# Autodesk Inventor assembly: Drivetrain 2025-2026
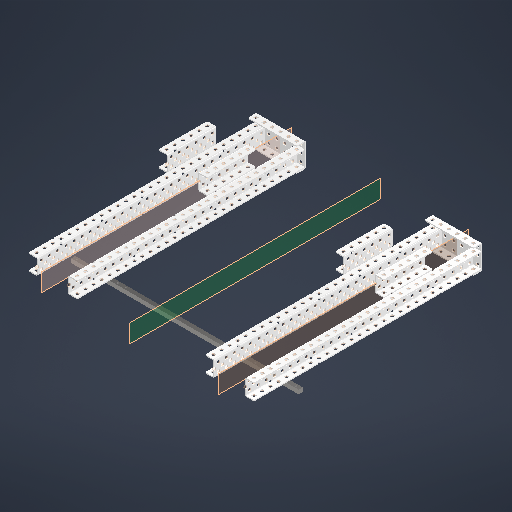
[picture p0: Inventor's stored thumbnail of the model, 512x512]
Saved by Autodesk Inventor 2026.2 (Build 302298000, 298)
## iProperties
Created: 2025-11-06
Part Number: Drivetrain 2025-2026
Document SubType Name: Assembly
Designer: thero
Author: thero
## Documents named in this file (12)
- C:\GitHub Repos\VEX-PushBack_2025-26\Push Back CAD\Drivetrain 2025-2026.iam
- C:\Users\thero\OneDrive\Desktop\VEX-CAD-Inventor-main\Structure\C Channel\Aluminum 1x2x1\Alu C 1x2x1x28.ipt
- C:\Users\thero\OneDrive\Desktop\VEX-CAD-Inventor-main\Structure\C Channel\Aluminum 1x2x1\Alu C 1x2x1x28_MIR.ipt
- C:\Users\thero\OneDrive\Desktop\VEX-CAD-Inventor-main\Structure\C Channel\Aluminum 1x3x1\Alu C 1x3x1x6.ipt
- C:\Users\thero\OneDrive\Desktop\VEX-CAD-Inventor-main\Structure\C Channel\Aluminum 1x2x1\Alu C 1x2x1x6.ipt
- C:\Users\thero\OneDrive\Desktop\VEX-CAD-Inventor-main\Structure\C Channel\Aluminum 1x2x1\Alu C 1x2x1x6_MIR.ipt
- C:\Users\thero\OneDrive\Desktop\VEX-CAD-Inventor-main\Structure\C Channel\Aluminum 1x2x1\Alu C 1x2x1x28_MIR1.ipt
- C:\Users\thero\OneDrive\Desktop\VEX-CAD-Inventor-main\Structure\C Channel\Aluminum 1x2x1\Alu C 1x2x1x28_MIR_MIR.ipt
- C:\Users\thero\OneDrive\Desktop\VEX-CAD-Inventor-main\Structure\C Channel\Aluminum 1x3x1\Alu C 1x3x1x6_MIR.ipt
- C:\Users\thero\OneDrive\Desktop\VEX-CAD-Inventor-main\Structure\C Channel\Aluminum 1x2x1\Alu C 1x2x1x6_MIR1.ipt
- C:\Users\thero\OneDrive\Desktop\VEX-CAD-Inventor-main\Structure\C Channel\Aluminum 1x2x1\Alu C 1x2x1x6_MIR_MIR.ipt
- C:\GitHub Repos\VEX-PushBack_2025-26\Push Back CAD\Chassis Cross Brace.ipt
## Components (11 placed, 11 different names)
1. Alu C 1x2x1x28:1 — Flush:1, Insert:1, Insert:3, Insert:4, Flush:2
2. Alu C 1x2x1x28_MIR:1 — Mate:1, Insert:2, Insert:9
3. Alu C 1x3x1x6:1 — Insert:1, Insert:2
4. Alu C 1x2x1x6:1 — Insert:3, Insert:4
5. Alu C 1x2x1x6_MIR:1
6. Alu C 1x2x1x28_MIR1:1 — Flush:3, Insert:6, Insert:7, Insert:8, Mate:3
7. Alu C 1x2x1x28_MIR_MIR:1 — Mate:2, Insert:5
8. Alu C 1x3x1x6_MIR:1 — Insert:5, Insert:6
9. Alu C 1x2x1x6_MIR1:1 — Insert:7, Insert:8
10. Alu C 1x2x1x6_MIR_MIR:1
11. Chassis Cross Brace:1 — Insert:9
## Relationships (15: Insert 9, Flush 3, Mate 3)
- Flush:1 (-38.1 mm): Alu C 1x2x1x28:1
- Mate:1 (-38.1 mm): Alu C 1x2x1x28_MIR:1
- Insert:1: Alu C 1x2x1x28:1 ↔ Alu C 1x3x1x6:1
- Insert:2: Alu C 1x2x1x28_MIR:1 ↔ Alu C 1x3x1x6:1
- Insert:3 (12.7 mm): Alu C 1x2x1x28:1 ↔ Alu C 1x2x1x6:1
- Insert:4 (12.7 mm): Alu C 1x2x1x28:1 ↔ Alu C 1x2x1x6:1
- Flush:2 (-114.3 mm): Alu C 1x2x1x28:1
- Flush:3 (-38.1 mm): Alu C 1x2x1x28_MIR1:1
- Mate:2 (-38.1 mm): Alu C 1x2x1x28_MIR_MIR:1
- Insert:5: Alu C 1x2x1x28_MIR_MIR:1 ↔ Alu C 1x3x1x6_MIR:1
- Insert:6: Alu C 1x2x1x28_MIR1:1 ↔ Alu C 1x3x1x6_MIR:1
- Insert:7 (12.7 mm): Alu C 1x2x1x28_MIR1:1 ↔ Alu C 1x2x1x6_MIR1:1
- Insert:8 (12.7 mm): Alu C 1x2x1x28_MIR1:1 ↔ Alu C 1x2x1x6_MIR1:1
- Mate:3 (-114.3 mm): Alu C 1x2x1x28_MIR1:1
- Insert:9 (15.875 mm): Alu C 1x2x1x28_MIR:1 ↔ Chassis Cross Brace:1
